# Autodesk Inventor assembly: linh2_mawts traau
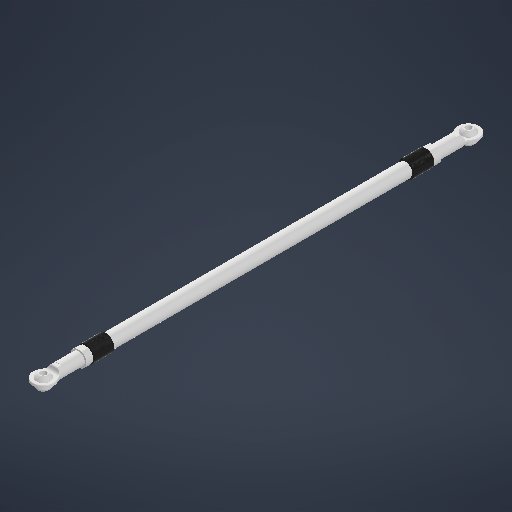
[picture p0: Inventor's stored thumbnail of the model, 512x512]
Saved by Autodesk Inventor 2027.1 (Build 311270010, 270A)
## iProperties
Created: 2026-08-18
Part Number: linh2_mawts traau
Document SubType Name: Assembly
Designer: MSI
Author: MSI
## Documents named in this file (5)
- C:\Users\MSI\Documents\MECHATRONICS\Tot_nghiep\Do_an_Delta.Robot_Dang_Rui_Bi\Thiết kế\Delta Part\linh2_mawts traau.iam
- C:\Users\MSI\Documents\MECHATRONICS\Tot_nghiep\Do_an_Delta.Robot_Dang_Rui_Bi\Thiết kế\Delta Part\link2.ipt
- C:\Users\MSI\Documents\MECHATRONICS\Tot_nghiep\Do_an_Delta.Robot_Dang_Rui_Bi\Thiết kế\Delta Part\khớp nối.ipt
- C:\Users\MSI\Documents\MECHATRONICS\Tot_nghiep\Do_an_Delta.Robot_Dang_Rui_Bi\Thiết kế\Delta Part\vòng bi_dài 35mm.ipt
- C:\Users\MSI\Documents\MECHATRONICS\Tot_nghiep\Do_an_Delta.Robot_Dang_Rui_Bi\Thiết kế\Delta Part\mắt trâu.ipt
## Components (7 placed, 4 different names)
1. link2:1 — Mate:1, Mate:2, Mate:3, Mate:4
2. khớp nối:1 — Mate:1, Mate:2, Mate:5, Mate:6
3. khớp nối:2 — Mate:3, Mate:4, Mate:7, Mate:8
4. vòng bi_dài 35mm:1 — Mate:5, Mate:6, Flush:1, Mate:11, Mate:12
5. vòng bi_dài 35mm:2 — Mate:7, Mate:8, Flush:1, Mate:9, Mate:10
6. mắt trâu:1 — Mate:11, Mate:12
7. mắt trâu:2 — Mate:9, Mate:10
## Relationships (13: Mate 12, Flush 1)
- Mate:1: link2:1 ↔ khớp nối:1
- Mate:2: link2:1 ↔ khớp nối:1
- Mate:3: link2:1 ↔ khớp nối:2
- Mate:4: link2:1 ↔ khớp nối:2
- Mate:5: khớp nối:1 ↔ vòng bi_dài 35mm:1
- Mate:6: khớp nối:1 ↔ vòng bi_dài 35mm:1
- Mate:7: khớp nối:2 ↔ vòng bi_dài 35mm:2
- Mate:8: khớp nối:2 ↔ vòng bi_dài 35mm:2
- Flush:1: vòng bi_dài 35mm:1 ↔ vòng bi_dài 35mm:2
- Mate:9: vòng bi_dài 35mm:2 ↔ mắt trâu:2
- Mate:10: vòng bi_dài 35mm:2 ↔ mắt trâu:2
- Mate:11: vòng bi_dài 35mm:1 ↔ mắt trâu:1
- Mate:12: vòng bi_dài 35mm:1 ↔ mắt trâu:1
